# Autodesk Inventor assembly: base_assembly
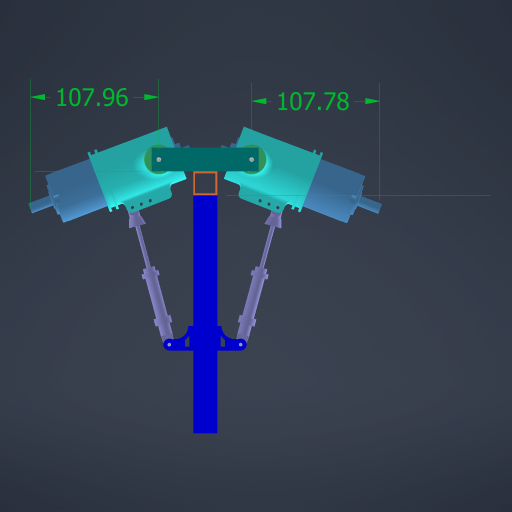
[picture p0: Inventor's stored thumbnail of the model, 512x512]
Saved by Autodesk Inventor 2024 (Build 280153000, 153)
## iProperties
Created: 2023-04-14
Part Number: base_assembly
Document SubType Name: Assembly
Designer: user
Author: user
## Documents named in this file (11)
- D:\Docs\Robot\3d\base\base_assembly.iam
- D:\Docs\Robot\3d\base\main axis.ipt
- D:\Docs\Robot\3d\base\section.ipt
- D:\Docs\Robot\3d\motor_assembly\side\motor_assembly_S.iam
- D:\Docs\Robot\3d\motor_assembly\side\motor_assembly_S_MIR.iam
- D:\Docs\Robot\3d\motor_assembly\midel\motor_assembly_M.iam
- D:\Docs\Robot\3d\default_components\shock_absorber.ipt
- D:\Docs\Robot\3d\machine_body\shock_absorber_holder_up.ipt
- C:\Users\user\Documents\Inventor\Content Center Files\R2024\ru-RU\DIN 7985 (H)\DIN 7985 (H) - M3x30-H.ipt
- D:\Docs\Robot\3d\base\shock_absorber_holder_down_150.ipt
- D:\Docs\Robot\3d\base\shock_absorber_holder_down_200.ipt
## Components (29 placed, 10 different names)
1. main axis:1 — Совмещение:1, Совмещение:2, Совмещение:8, Плоский:1, Плоский:5, Плоский:6, Плоский:8, Совмещение:37, Совмещение:38, Совмещение:41
2. section:1 — Совмещение:1, Совмещение:2, Вставка:2, Вставка:3, Совмещение:46
3. section:3 — Вставка:4, Вставка:5, Вставка:6, Вставка:7
4. motor_assembly_M:1 [sub-assembly] — Вставка:6, Вставка:9, Цилиндрический:10, Совмещение:31
5. motor_assembly_M:2 [sub-assembly] — Вставка:7, Вставка:8, Цилиндрический:9, Совмещение:32
6. motor_assembly_S:1 [sub-assembly] — Вставка:3, Вставка:5, Цилиндрический:3, Совмещение:29
7. motor_assembly_S_MIR:1 [sub-assembly] — Вставка:2, Вставка:4, Цилиндрический:4, Совмещение:28
8. section:4 — Вставка:8, Вставка:9, Вставка:10, Вставка:14
9. section:5 — Вставка:13, Вставка:15, Совмещение:45, Совмещение:47
10. motor_assembly_S:2 [sub-assembly] — Вставка:10, Вставка:13, Цилиндрический:11, Совмещение:33
11. motor_assembly_S_MIR:2 [sub-assembly] — Вставка:14, Вставка:15, Цилиндрический:12, Совмещение:30
12. shock_absorber_holder_up:1 — Вставка:20, Вставка:23, Плоский:9, Совмещение:35, Совмещение:36, Совмещение:50
13. shock_absorber_holder_up:2 — Вставка:21, Вставка:24, Совмещение:39, Совмещение:40, Плоский:10, Совмещение:51
14. shock_absorber_holder_up:3 — Вставка:22, Вставка:25, Плоский:4, Плоский:7, Совмещение:34, Совмещение:48
15. DIN 7985 (H) M3x30-H:1 — Вставка:20, Цилиндрический:7
16. DIN 7985 (H) M3x30-H:2 — Вставка:21, Цилиндрический:8
17. DIN 7985 (H) M3x30-H:3 — Вставка:22, Цилиндрический:1
18. DIN 7985 (H) M3x30-H:4 — Вставка:24, Цилиндрический:5
19. DIN 7985 (H) M3x30-H:5 — Вставка:23, Цилиндрический:6
20. DIN 7985 (H) M3x30-H:6 — Вставка:25, Цилиндрический:2
21. shock_absorber:1 — Цилиндрический:5, Цилиндрический:10, Совмещение:31, Плоский:10
22. shock_absorber:2 — Цилиндрический:2, Цилиндрический:3, Совмещение:29, Плоский:4
23. shock_absorber:3 — Цилиндрический:1, Цилиндрический:4, Совмещение:28
24. shock_absorber:4 — Цилиндрический:6, Цилиндрический:12, Совмещение:30, Плоский:9
25. shock_absorber:5 — Цилиндрический:7, Цилиндрический:11, Совмещение:33
26. shock_absorber:6 — Цилиндрический:8, Цилиндрический:9, Совмещение:32
27. shock_absorber_holder_down_150:1 — Плоский:1, Плоский:8, Совмещение:35, Совмещение:36, Совмещение:37, Совмещение:50
28. shock_absorber_holder_down_150:2 — Плоский:5, Плоский:6, Плоский:7, Совмещение:34, Совмещение:48
29. shock_absorber_holder_down_200:1 — Совмещение:38, Совмещение:39, Совмещение:40, Совмещение:41, Совмещение:51
## Relationships (62: Mate 23, Insert 18, CylindricalJoint 12, PlanarJoint 8, Angle 1)
- Совмещение:1 [Mate]: main axis:1 ↔ section:1
- Совмещение:2 [Mate] (55 mm): main axis:1 ↔ section:1
- Вставка:2 [Insert]: section:1 ↔ motor_assembly_S_MIR:1
- Вставка:3 [Insert]: section:1 ↔ motor_assembly_S:1
- Вставка:4 [Insert]: section:3 ↔ motor_assembly_S_MIR:1
- Вставка:5 [Insert]: section:3 ↔ motor_assembly_S:1
- Вставка:6 [Insert]: section:3 ↔ motor_assembly_M:1
- Вставка:7 [Insert]: section:3 ↔ motor_assembly_M:2
- Вставка:8 [Insert]: motor_assembly_M:2 ↔ section:4
- Вставка:9 [Insert]: motor_assembly_M:1 ↔ section:4
- Вставка:10 [Insert]: section:4 ↔ motor_assembly_S:2
- Вставка:13 [Insert]: section:5 ↔ motor_assembly_S:2
- Вставка:14 [Insert]: section:4 ↔ motor_assembly_S_MIR:2
- Вставка:15 [Insert]: section:5 ↔ motor_assembly_S_MIR:2
- Совмещение:8 [Mate]: main axis:1
- Угол:2 [Angle] (0 deg)
- Вставка:20 [Insert]: shock_absorber_holder_up:1 ↔ DIN 7985 (H) M3x30-H:1
- Вставка:21 [Insert]: shock_absorber_holder_up:2 ↔ DIN 7985 (H) M3x30-H:2
- Вставка:22 [Insert]: shock_absorber_holder_up:3 ↔ DIN 7985 (H) M3x30-H:3
- Вставка:23 [Insert]: shock_absorber_holder_up:1 ↔ DIN 7985 (H) M3x30-H:5
- Вставка:24 [Insert]: shock_absorber_holder_up:2 ↔ DIN 7985 (H) M3x30-H:4
- Вставка:25 [Insert]: shock_absorber_holder_up:3 ↔ DIN 7985 (H) M3x30-H:6
- Цилиндрический:1 [CylindricalJoint]: DIN 7985 (H) M3x30-H:3 ↔ shock_absorber:3
- Цилиндрический:2 [CylindricalJoint]: DIN 7985 (H) M3x30-H:6 ↔ shock_absorber:2
- Цилиндрический:3 [CylindricalJoint]: motor_assembly_S:1 ↔ shock_absorber:2
- Цилиндрический:4 [CylindricalJoint]: motor_assembly_S_MIR:1 ↔ shock_absorber:3
- Цилиндрический:5 [CylindricalJoint]: DIN 7985 (H) M3x30-H:4 ↔ shock_absorber:1
- Совмещение:28 [Mate]: motor_assembly_S_MIR:1 ↔ shock_absorber:3
- Совмещение:29 [Mate]: motor_assembly_S:1 ↔ shock_absorber:2
- Цилиндрический:6 [CylindricalJoint]: DIN 7985 (H) M3x30-H:5 ↔ shock_absorber:4
- Цилиндрический:7 [CylindricalJoint]: DIN 7985 (H) M3x30-H:1 ↔ shock_absorber:5
- Цилиндрический:8 [CylindricalJoint]: DIN 7985 (H) M3x30-H:2 ↔ shock_absorber:6
- Цилиндрический:9 [CylindricalJoint]: motor_assembly_M:2 ↔ shock_absorber:6
- Цилиндрический:10 [CylindricalJoint]: motor_assembly_M:1 ↔ shock_absorber:1
- Цилиндрический:11 [CylindricalJoint]: motor_assembly_S:2 ↔ shock_absorber:5
- Цилиндрический:12 [CylindricalJoint]: motor_assembly_S_MIR:2 ↔ shock_absorber:4
- Совмещение:30 [Mate]: motor_assembly_S_MIR:2 ↔ shock_absorber:4
- Совмещение:31 [Mate]: motor_assembly_M:1 ↔ shock_absorber:1
- Совмещение:32 [Mate]: motor_assembly_M:2 ↔ shock_absorber:6
- Совмещение:33 [Mate]: motor_assembly_S:2 ↔ shock_absorber:5
- Плоский:1 [PlanarJoint]: main axis:1 ↔ shock_absorber_holder_down_150:1
- Плоский:4 [PlanarJoint] (5 mm): shock_absorber_holder_up:3 ↔ shock_absorber:2
- Плоский:5 [PlanarJoint]: main axis:1 ↔ shock_absorber_holder_down_150:2
- Плоский:6 [PlanarJoint]: main axis:1 ↔ shock_absorber_holder_down_150:2
- Плоский:7 [PlanarJoint]: shock_absorber_holder_up:3 ↔ shock_absorber_holder_down_150:2
- Совмещение:34 [Mate]: shock_absorber_holder_up:3 ↔ shock_absorber_holder_down_150:2
- Плоский:8 [PlanarJoint]: main axis:1 ↔ shock_absorber_holder_down_150:1
- Плоский:9 [PlanarJoint] (5 mm): shock_absorber_holder_up:1 ↔ shock_absorber:4
- Совмещение:35 [Mate]: shock_absorber_holder_up:1 ↔ shock_absorber_holder_down_150:1
- Совмещение:36 [Mate]: shock_absorber_holder_up:1 ↔ shock_absorber_holder_down_150:1
- Совмещение:37 [Mate]: main axis:1 ↔ shock_absorber_holder_down_150:1
- Совмещение:38 [Mate]: main axis:1 ↔ shock_absorber_holder_down_200:1
- Совмещение:39 [Mate]: shock_absorber_holder_up:2 ↔ shock_absorber_holder_down_200:1
- Совмещение:40 [Mate]: shock_absorber_holder_up:2 ↔ shock_absorber_holder_down_200:1
- Плоский:10 [PlanarJoint] (5 mm): shock_absorber_holder_up:2 ↔ shock_absorber:1
- Совмещение:41 [Mate]: main axis:1 ↔ shock_absorber_holder_down_200:1
- Совмещение:45 [Mate]: section:5
- Совмещение:46 [Mate]: section:1
- Совмещение:47 [Mate]: section:5
- Совмещение:48 [Mate] (20 mm): shock_absorber_holder_up:3 ↔ shock_absorber_holder_down_150:2
- Совмещение:50 [Mate] (20 mm): shock_absorber_holder_up:1 ↔ shock_absorber_holder_down_150:1
- Совмещение:51 [Mate] (70 mm): shock_absorber_holder_up:2 ↔ shock_absorber_holder_down_200:1
## Named parameters: hw = 1 mm, up_sh = 20 mm
